# Autodesk Inventor assembly: Сборка
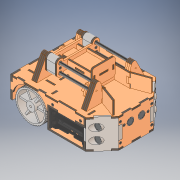
[picture p0: Inventor's stored thumbnail of the model, 180x180]
Saved by Autodesk Inventor 2019 (Build 230136000, 136)
## iProperties
Created: 2020-12-06
Part Number: Сборка
Material: Типовые
Document SubType Name: Assembly
Designer: Professional
Author: Professional
## Documents named in this file (51)
- C:\Users\Professional\Documents\DeliveryBot\3dModels\assembly.iam
- C:\Users\Professional\Documents\DeliveryBot\3dModels\Components\42BYGH47.ipt
- C:\Users\Professional\Documents\DeliveryBot\3dModels\LaserCutter\base.ipt
- C:\Users\Professional\Documents\DeliveryBot\3dModels\LaserCutter\top.ipt
- C:\Users\Professional\Documents\DeliveryBot\3dModels\LaserCutter\batTop.ipt
- C:\Users\Professional\Documents\DeliveryBot\3dModels\3DPrinter\Sensor_L.ipt
- C:\Users\Professional\Documents\DeliveryBot\3dModels\LaserCutter\batMain.ipt
- C:\Users\Professional\Documents\DeliveryBot\3dModels\LaserCutter\batBack.ipt
- C:\Users\Professional\Documents\DeliveryBot\3dModels\LaserCutter\batN.ipt
- C:\Users\Professional\Documents\DeliveryBot\3dModels\LaserCutter\spacer.ipt
- C:\Users\Professional\Documents\DeliveryBot\3dModels\LaserCutter\stepperMount.ipt
- C:\Users\Professional\Documents\DeliveryBot\3dModels\LaserCutter\stiffenerFront.ipt
- C:\Users\Professional\Documents\DeliveryBot\3dModels\LaserCutter\stiffenerBack.ipt
- C:\Users\Professional\Documents\DeliveryBot\3dModels\3DPrinter\sameSpacer.ipt
- C:\Users\Professional\Documents\DeliveryBot\3dModels\LaserCutter\back.ipt
- C:\Users\Professional\Documents\DeliveryBot\3dModels\3DPrinter\wheel_L.ipt
- C:\Users\Professional\Documents\DeliveryBot\3dModels\3DPrinter\wheel_R.ipt
- C:\Users\Professional\Documents\DeliveryBot\3dModels\LaserCutter\protector.ipt
- C:\Users\Professional\Documents\DeliveryBot\3dModels\components\HC-SR04.ipt
- C:\Users\Professional\Documents\DeliveryBot\3dModels\components\CNC shield.ipt
- C:\Users\Professional\Documents\DeliveryBot\3dModels\Components\2x18650 holder.ipt
- C:\Users\Professional\Documents\DeliveryBot\3dModels\components\smallWheel.ipt
- C:\Users\Professional\Documents\DeliveryBot\3dModels\3DPrinter\smallWheelStator.ipt
- C:\Users\Professional\Documents\DeliveryBot\3dModels\3DPrinter\CupHolder.ipt
- C:\Users\Professional\Documents\DeliveryBot\3dModels\Components\LineSensor.ipt
- C:\Users\Professional\Documents\DeliveryBot\3dModels\3DPrinter\StructureCenter.ipt
- C:\Users\Professional\Documents\DeliveryBot\3dModels\3DPrinter\CupHolderBack.ipt
- C:\Users\Professional\Documents\DeliveryBot\3dModels\3DPrinter\Sensor_R.ipt
- C:\Users\Professional\Documents\DeliveryBot\3dModels\LaserCutter\ElectronicPlate.ipt
- C:\Users\Professional\Documents\DeliveryBot\3dModels\Components\DC-DC sown.ipt
- C:\Users\Professional\Documents\DeliveryBot\3dModels\Fasteners\M3x16P.ipt
- C:\Users\Professional\Documents\DeliveryBot\3dModels\Fasteners\M3x10P.ipt
- C:\Users\Professional\Documents\DeliveryBot\3dModels\3DPrinter\FrontSensor.ipt
- C:\Users\Professional\Documents\DeliveryBot\3dModels\Components\ArduinoMega.ipt
- C:\Users\Professional\Documents\DeliveryBot\3dModels\LaserCutter\HolderDCDC.ipt
- C:\Users\Professional\Documents\DeliveryBot\3dModels\LaserCutter\stiffenerDCDC.ipt
- C:\Users\Professional\Documents\DeliveryBot\3dModels\Fasteners\M3_MF_6mm.ipt
- C:\Users\Professional\Documents\DeliveryBot\3dModels\LaserCutter\topCase.ipt
- C:\Users\Professional\Documents\DeliveryBot\3dModels\Components\SFC6.ipt
- C:\Users\Professional\Documents\DeliveryBot\3dModels\Components\LM6UU.ipt
- C:\Users\Professional\Documents\DeliveryBot\3dModels\LaserCutter\HolderSFC6.ipt
- C:\Users\Professional\Documents\DeliveryBot\3dModels\LaserCutter\StopperSFC6.ipt
- C:\Users\Professional\Documents\DeliveryBot\3dModels\LaserCutter\PistonPart1.ipt
- C:\Users\Professional\Documents\DeliveryBot\3dModels\LaserCutter\PistonPart2.ipt
- C:\Users\Professional\Documents\DeliveryBot\3dModels\LaserCutter\PistonPart3.ipt
- C:\Users\Professional\Documents\DeliveryBot\3dModels\LaserCutter\PistonPart4.ipt
- C:\Users\Professional\Documents\DeliveryBot\3dModels\LaserCutter\PistonPart5.ipt
- C:\Users\Professional\Documents\DeliveryBot\3dModels\3DPrinter\BearingIn.ipt
- C:\Users\Professional\Documents\DeliveryBot\3dModels\LaserCutter\Limiter1.ipt
- C:\Users\Professional\Documents\DeliveryBot\3dModels\LaserCutter\Limiter2.ipt
- C:\Users\Professional\Documents\DeliveryBot\3dModels\LaserCutter\Limiter3.ipt
## Components (164 placed, 50 different names)
1. 42BYGH47:1 — Угол:1, Жесткий:24, С поворотом:2
2. base:1 — Жесткий:1, Жесткий:4, Жесткий:6, Жесткий:8, Жесткий:9, Жесткий:10, Жесткий:11, Жесткий:12, Жесткий:18, Жесткий:19, Жесткий:22, Жесткий:23, Жесткий:37, Жесткий:38, Жесткий:45, Жесткий:46, С поворотом:4, С поворотом:5, С поворотом:31, С поворотом:32, С поворотом:33, С поворотом:34, С поворотом:65, С поворотом:74, С поворотом:75, С поворотом:76, С поворотом:77, С поворотом:90, С поворотом:91, С поворотом:92, С поворотом:93, С поворотом:94, С поворотом:95, С поворотом:96, С поворотом:97
3. top:1 — Жесткий:1, С поворотом:70, С поворотом:71, С поворотом:72, С поворотом:73, Жесткий:64, Жесткий:80, Жесткий:81, Жесткий:82
4. 42BYGH47:2 — Угол:1, Жесткий:25, С поворотом:1
5. batTop:1 — Жесткий:8, Жесткий:13, С поворотом:69
6. batTop:2 — Жесткий:4, Жесткий:15, Жесткий:51, С поворотом:10
7. Sensor_L:2 — Жесткий:6, Жесткий:33
8. batMain:1 — Жесткий:10, Жесткий:35
9. batMain:2 — Жесткий:9, Жесткий:53, Угол:4
10. batBack:1 — Жесткий:11, С поворотом:66
11. batBack:2 — Жесткий:12, С поворотом:9
12. batN:1 — Жесткий:13, Жесткий:16
13. batN:2 — Жесткий:15, Жесткий:28
14. spacer:1 — Жесткий:16, Жесткий:40, С поворотом:67, С поворотом:68
15. stepperMount:1 — Жесткий:19, Жесткий:24, С поворотом:27, С поворотом:28, С поворотом:29, С поворотом:30, С поворотом:78, С поворотом:79, С поворотом:80, С поворотом:81
16. stepperMount:2 — Жесткий:18, Жесткий:25, С поворотом:19, С поворотом:20, С поворотом:21, С поворотом:22, С поворотом:82, С поворотом:83, С поворотом:84, С поворотом:85
17. stiffenerFront:1 — Жесткий:22, Жесткий:47, Жесткий:48, С поворотом:15, С поворотом:16, С поворотом:17, С поворотом:18
18. stiffenerBack:1 — Жесткий:23, Жесткий:31, Жесткий:49, Жесткий:50, С поворотом:11, С поворотом:12, С поворотом:13, С поворотом:14
19. back:1 — Жесткий:29, Жесткий:30, Жесткий:39, С поворотом:23, С поворотом:24, С поворотом:25, С поворотом:26
20. wheel_L:2 — С поворотом:1
21. wheel_R:1 — С поворотом:2
22. spacer:2 — Жесткий:28, Жесткий:41, Жесткий:63, С поворотом:8
23. protector:1 — Жесткий:29
24. protector:2 — Жесткий:30
25. sameSpacer:1 — Жесткий:31, Жесткий:39
26. smallWheel:1 — С поворотом:3
27. smallWheelStator:1 — Жесткий:38, С поворотом:98
28. smallWheelStator:2 — Жесткий:37, С поворотом:3
29. CupHolder:1 — Жесткий:41
30. CupHolder:2 — Жесткий:40
31. StructureCenter:1 — Жесткий:48
32. StructureCenter:2 — Жесткий:47, Цилиндрический:1
33. CupHolderBack:1 — Жесткий:50
34. CupHolderBack:2 — Жесткий:49
35. Sensor_R:1 — Жесткий:51, Жесткий:52
36. FrontSensor:1 — Жесткий:64, Жесткий:65
37. topCase:1 — Жесткий:82, Жесткий:83, Жесткий:87, Жесткий:90, Жесткий:91, Угол:7, Угол:8, Жесткий:111, Жесткий:112, Жесткий:113, Жесткий:114, Жесткий:115
38. SFC6:1 — Жесткий:86, Цилиндрический:2
39. LM6UU:2 — Цилиндрический:2, Заподлицо:2
40. HolderSFC6:1 — Жесткий:83, Жесткий:84
41. HolderSFC6:2 — Жесткий:84, Жесткий:85, Жесткий:86, Жесткий:96
42. StopperSFC6:1 — Жесткий:85
43. StopperSFC6:3 — Жесткий:90, Жесткий:94
44. StopperSFC6:4 — Жесткий:87, Жесткий:88
45. HolderSFC6:3 — Жесткий:88, Жесткий:89
46. HolderSFC6:4 — Жесткий:89
47. StopperSFC6:5 — Жесткий:91, Жесткий:92
48. HolderSFC6:6 — Жесткий:92, Жесткий:93, Жесткий:97, Жесткий:98
49. HolderSFC6:7 — Жесткий:93
50. HolderSFC6:8 — Жесткий:95
51. HolderSFC6:9 — Жесткий:94, Жесткий:95
52. SFC6:4 — Жесткий:96
53. LM6UU:3 — Заподлицо:2, Заподлицо:3, Жесткий:99, Жесткий:105
54. SFC6:5 — Жесткий:98
55. LM6UU:4 — Заподлицо:1, Заподлицо:3, С поворотом:101
56. SFC6:6 — Жесткий:97
57. LM6UU:5 — Заподлицо:1
58. PistonPart1:1 — Жесткий:99, Угол:7, Жесткий:104, Жесткий:106, Жесткий:107, Жесткий:108
59. PistonPart2:1 — С поворотом:101, Угол:8, Жесткий:109, Жесткий:110
60. PistonPart3:1 — Жесткий:101, Жесткий:102, Жесткий:103, Жесткий:104
61. PistonPart4:1 — Жесткий:102
62. PistonPart4:2 — Жесткий:101
63. PistonPart5:1 — Жесткий:103
64. BearingIn:1 — Жесткий:106
65. BearingIn:2 — Жесткий:105
66. M3x10P:52 — Жесткий:107
67. M3x10P:53 — Жесткий:108
68. M3x10P:54 — Жесткий:109
69. M3x10P:55 — Жесткий:110
70. Limiter1:1 — Жесткий:111
71. Limiter1:2 — Жесткий:112
72. Limiter2:1 — Жесткий:113
73. Limiter3:1 — Жесткий:115
74. Limiter3:2 — Жесткий:114
75. M3x10P:42 — С поворотом:90
76. M3x10P:43 — С поворотом:92
77. M3x10P:44 — С поворотом:91
78. M3x10P:45 — С поворотом:93
79. M3x10P:46 — С поворотом:97
80. M3x10P:47 — С поворотом:94
81. M3x10P:48 — С поворотом:96
82. M3x10P:49 — С поворотом:95
83. M3x16P:16 — С поворотом:98
84. M3x10P:50 — Жесткий:80
85. M3x10P:51 — Жесткий:81
86. M3x16P:2 — С поворотом:8
87. M3x16P:3 — С поворотом:9
88. M3x16P:5 — С поворотом:10
89. M3x16P:6 — С поворотом:14
90. M3x16P:7 — С поворотом:13
91. M3x16P:8 — С поворотом:12
92. M3x16P:11 — С поворотом:11
93. M3x10P:2 — С поворотом:16
94. M3x10P:3 — С поворотом:17
95. M3x10P:4 — С поворотом:15
96. M3x10P:5 — С поворотом:21
97. M3x10P:6 — С поворотом:29
98. M3x10P:7 — С поворотом:23
99. M3x10P:8 — С поворотом:22
100. M3x10P:9 — С поворотом:27
101. M3x10P:10 — С поворотом:28
102. M3x10P:11 — С поворотом:19
103. M3x10P:12 — С поворотом:30
104. M3x10P:13 — С поворотом:31
105. M3x10P:14 — С поворотом:20
106. M3x10P:15 — С поворотом:26
107. M3x10P:16 — С поворотом:24
108. M3x10P:17 — С поворотом:25
109. M3x10P:18 — С поворотом:32
110. M3x10P:19 — С поворотом:34
111. M3x10P:20 — С поворотом:33
112. M3x10P:21 — С поворотом:65
113. M3x16P:12 — С поворотом:68
114. M3x16P:13 — С поворотом:67
115. M3x16P:14 — С поворотом:69
116. M3x16P:15 — С поворотом:66
117. M3x10P:22 — С поворотом:73
118. M3x10P:23 — С поворотом:72
119. M3x10P:24 — С поворотом:71
120. M3x10P:25 — С поворотом:70
121. M3x10P:26 — С поворотом:74
122. M3x10P:27 — С поворотом:75
123. M3x10P:28 — С поворотом:76
124. M3x10P:29 — С поворотом:77
125. M3x10P:30 — С поворотом:81
126. M3x10P:31 — С поворотом:80
127. M3x10P:32 — С поворотом:79
128. M3x10P:33 — С поворотом:78
129. M3x10P:34 — С поворотом:82
130. M3x10P:35 — С поворотом:83
131. M3x10P:36 — С поворотом:84
132. M3x10P:37 — С поворотом:85
133. M3x10P:1 — С поворотом:18
134. M3x16P:1 — Жесткий:63
135. HolderDCDC:1 — Жесткий:66, Жесткий:67, Жесткий:68, Жесткий:69, Жесткий:70, Жесткий:71, Жесткий:72
136. stiffenerDCDC:1 — Жесткий:67
137. stiffenerDCDC:2 — Жесткий:68
138. DC-DC sown:1 — Жесткий:73
139. ArduinoMega:1 — С поворотом:99, Угол:5, С поворотом:100, Угол:6
140. CNC shield:1 — С поворотом:100, Угол:6
141. ElectronicPlate:1 — Цилиндрический:1, С поворотом:86, С поворотом:87, С поворотом:88, С поворотом:89, Жесткий:66, Угол:4, Жесткий:74, Жесткий:75, Жесткий:76, Жесткий:77, Жесткий:78, Жесткий:79, Угол:5
142. M3x10P:38 — С поворотом:87
143. M3x10P:39 — С поворотом:89
144. M3x10P:40 — С поворотом:88
145. M3x10P:41 — С поворотом:86
146. M3_MF_6mm:1 — Жесткий:69, Жесткий:73
147. M3_MF_6mm:2 — Жесткий:70
148. M3_MF_6mm:3 — Жесткий:72
149. M3_MF_6mm:4 — Жесткий:71
150. M3_MF_6mm:5 — Жесткий:76
151. M3_MF_6mm:6 — Жесткий:75
152. M3_MF_6mm:7 — Жесткий:77
153. M3_MF_6mm:8 — Жесткий:78
154. M3_MF_6mm:9 — Жесткий:74, С поворотом:99
155. M3_MF_6mm:10 — Жесткий:79
156. 2x18650 holder:2 — Жесткий:53
157. HC-SR04:2 — Жесткий:52
158. HC-SR04:1 — Жесткий:33
159. 2x18650 holder:1 — Жесткий:35
160. LineSensor:4 — С поворотом:4
161. LineSensor:3 — С поворотом:5
162. LineSensor:2 — Жесткий:45
163. LineSensor:1 — Жесткий:46
164. HC-SR04:3 — Жесткий:65
## Relationships (172: WeldJoint 89, RevoluteJoint 69, Angle 6, CylindricalJoint 5, Flush 3)
- Жесткий:1 [WeldJoint]: base:1 ↔ top:1
- Угол:1 [Angle] (180 deg): 42BYGH47:1 ↔ 42BYGH47:2
- Жесткий:4 [WeldJoint]: base:1 ↔ batTop:2
- Жесткий:6 [WeldJoint]: base:1 ↔ Sensor_L:2
- Жесткий:8 [WeldJoint]: base:1 ↔ batTop:1
- Жесткий:9 [WeldJoint]: base:1 ↔ batMain:2
- Жесткий:10 [WeldJoint]: base:1 ↔ batMain:1
- Жесткий:11 [WeldJoint]: base:1 ↔ batBack:1
- Жесткий:12 [WeldJoint]: base:1 ↔ batBack:2
- Жесткий:13 [WeldJoint]: batTop:1 ↔ batN:1
- Жесткий:15 [WeldJoint]: batTop:2 ↔ batN:2
- Жесткий:16 [WeldJoint]: batN:1 ↔ spacer:1
- Жесткий:18 [WeldJoint]: base:1 ↔ stepperMount:2
- Жесткий:19 [WeldJoint]: base:1 ↔ stepperMount:1
- Жесткий:22 [WeldJoint]: base:1 ↔ stiffenerFront:1
- Жесткий:23 [WeldJoint]: base:1 ↔ stiffenerBack:1
- Жесткий:24 [WeldJoint]: 42BYGH47:1 ↔ stepperMount:1
- Жесткий:25 [WeldJoint]: 42BYGH47:2 ↔ stepperMount:2
- С поворотом:1 [RevoluteJoint] (-19 mm): 42BYGH47:2 ↔ wheel_L:2
- С поворотом:2 [RevoluteJoint] (-19 mm): 42BYGH47:1 ↔ wheel_R:1
- Жесткий:28 [WeldJoint]: batN:2 ↔ spacer:2
- Жесткий:29 [WeldJoint]: back:1 ↔ protector:1
- Жесткий:30 [WeldJoint]: back:1 ↔ protector:2
- Жесткий:31 [WeldJoint]: stiffenerBack:1 ↔ sameSpacer:1
- Жесткий:33 [WeldJoint]: Sensor_L:2 ↔ HC-SR04:1
- Жесткий:35 [WeldJoint]: batMain:1 ↔ 2x18650 holder:1
- Жесткий:37 [WeldJoint]: base:1 ↔ smallWheelStator:2
- Жесткий:38 [WeldJoint]: base:1 ↔ smallWheelStator:1
- С поворотом:3 [RevoluteJoint]: smallWheel:1 ↔ smallWheelStator:2
- Жесткий:39 [WeldJoint]: back:1 ↔ sameSpacer:1
- Жесткий:40 [WeldJoint]: spacer:1 ↔ CupHolder:2
- Жесткий:41 [WeldJoint]: spacer:2 ↔ CupHolder:1
- Жесткий:45 [WeldJoint]: base:1 ↔ LineSensor:2
- Жесткий:46 [WeldJoint]: base:1 ↔ LineSensor:1
- С поворотом:4 [RevoluteJoint]: base:1 ↔ LineSensor:4
- С поворотом:5 [RevoluteJoint]: base:1 ↔ LineSensor:3
- Жесткий:47 [WeldJoint]: stiffenerFront:1 ↔ StructureCenter:2
- Жесткий:48 [WeldJoint]: stiffenerFront:1 ↔ StructureCenter:1
- Жесткий:49 [WeldJoint]: stiffenerBack:1 ↔ CupHolderBack:2
- Жесткий:50 [WeldJoint]: stiffenerBack:1 ↔ CupHolderBack:1
- Жесткий:51 [WeldJoint]: batTop:2 ↔ Sensor_R:1
- Жесткий:52 [WeldJoint]: Sensor_R:1 ↔ HC-SR04:2
- Жесткий:53 [WeldJoint]: batMain:2 ↔ 2x18650 holder:2
- Цилиндрический:1 [CylindricalJoint]: StructureCenter:2 ↔ ElectronicPlate:1
- Жесткий:63 [WeldJoint]: spacer:2 ↔ M3x16P:1
- С поворотом:8 [RevoluteJoint]: spacer:2 ↔ M3x16P:2
- С поворотом:9 [RevoluteJoint]: batBack:2 ↔ M3x16P:3
- С поворотом:10 [RevoluteJoint]: batTop:2 ↔ M3x16P:5
- С поворотом:11 [RevoluteJoint]: stiffenerBack:1 ↔ M3x16P:11
- С поворотом:12 [RevoluteJoint]: stiffenerBack:1 ↔ M3x16P:8
- С поворотом:13 [RevoluteJoint]: stiffenerBack:1 ↔ M3x16P:7
- С поворотом:14 [RevoluteJoint]: stiffenerBack:1 ↔ M3x16P:6
- С поворотом:15 [RevoluteJoint]: stiffenerFront:1 ↔ M3x10P:4
- С поворотом:16 [RevoluteJoint]: stiffenerFront:1 ↔ M3x10P:2
- С поворотом:17 [RevoluteJoint]: stiffenerFront:1 ↔ M3x10P:3
- С поворотом:18 [RevoluteJoint]: stiffenerFront:1 ↔ M3x10P:1
- С поворотом:19 [RevoluteJoint]: stepperMount:2 ↔ M3x10P:11
- С поворотом:20 [RevoluteJoint]: stepperMount:2 ↔ M3x10P:14
- С поворотом:21 [RevoluteJoint]: stepperMount:2 ↔ M3x10P:5
- С поворотом:22 [RevoluteJoint]: stepperMount:2 ↔ M3x10P:8
- С поворотом:23 [RevoluteJoint]: back:1 ↔ M3x10P:7
- С поворотом:24 [RevoluteJoint]: back:1 ↔ M3x10P:16
- С поворотом:25 [RevoluteJoint]: back:1 ↔ M3x10P:17
- С поворотом:26 [RevoluteJoint]: back:1 ↔ M3x10P:15
- С поворотом:27 [RevoluteJoint]: stepperMount:1 ↔ M3x10P:9
- С поворотом:28 [RevoluteJoint]: stepperMount:1 ↔ M3x10P:10
- С поворотом:29 [RevoluteJoint]: stepperMount:1 ↔ M3x10P:6
- С поворотом:30 [RevoluteJoint]: stepperMount:1 ↔ M3x10P:12
- С поворотом:31 [RevoluteJoint]: base:1 ↔ M3x10P:13
- С поворотом:32 [RevoluteJoint]: base:1 ↔ M3x10P:18
- С поворотом:33 [RevoluteJoint]: base:1 ↔ M3x10P:20
- С поворотом:34 [RevoluteJoint]: base:1 ↔ M3x10P:19
- С поворотом:65 [RevoluteJoint]: base:1 ↔ M3x10P:21
- С поворотом:66 [RevoluteJoint]: batBack:1 ↔ M3x16P:15
- С поворотом:67 [RevoluteJoint]: spacer:1 ↔ M3x16P:13
- С поворотом:68 [RevoluteJoint]: spacer:1 ↔ M3x16P:12
- С поворотом:69 [RevoluteJoint]: batTop:1 ↔ M3x16P:14
- С поворотом:70 [RevoluteJoint]: top:1 ↔ M3x10P:25
- С поворотом:71 [RevoluteJoint]: top:1 ↔ M3x10P:24
- С поворотом:72 [RevoluteJoint]: top:1 ↔ M3x10P:23
- С поворотом:73 [RevoluteJoint]: top:1 ↔ M3x10P:22
- С поворотом:74 [RevoluteJoint]: base:1 ↔ M3x10P:26
- С поворотом:75 [RevoluteJoint]: base:1 ↔ M3x10P:27
- С поворотом:76 [RevoluteJoint]: base:1 ↔ M3x10P:28
- С поворотом:77 [RevoluteJoint]: base:1 ↔ M3x10P:29
- С поворотом:78 [RevoluteJoint]: stepperMount:1 ↔ M3x10P:33
- С поворотом:79 [RevoluteJoint]: stepperMount:1 ↔ M3x10P:32
- С поворотом:80 [RevoluteJoint]: stepperMount:1 ↔ M3x10P:31
- С поворотом:81 [RevoluteJoint]: stepperMount:1 ↔ M3x10P:30
- С поворотом:82 [RevoluteJoint]: stepperMount:2 ↔ M3x10P:34
- С поворотом:83 [RevoluteJoint]: stepperMount:2 ↔ M3x10P:35
- С поворотом:84 [RevoluteJoint]: stepperMount:2 ↔ M3x10P:36
- С поворотом:85 [RevoluteJoint]: stepperMount:2 ↔ M3x10P:37
- С поворотом:86 [RevoluteJoint]: ElectronicPlate:1 ↔ M3x10P:41
- С поворотом:87 [RevoluteJoint]: ElectronicPlate:1 ↔ M3x10P:38
- С поворотом:88 [RevoluteJoint]: ElectronicPlate:1 ↔ M3x10P:40
- С поворотом:89 [RevoluteJoint]: ElectronicPlate:1 ↔ M3x10P:39
- С поворотом:90 [RevoluteJoint]: base:1 ↔ M3x10P:42
- С поворотом:91 [RevoluteJoint]: base:1 ↔ M3x10P:44
- С поворотом:92 [RevoluteJoint]: base:1 ↔ M3x10P:43
- С поворотом:93 [RevoluteJoint]: base:1 ↔ M3x10P:45
- С поворотом:94 [RevoluteJoint]: base:1 ↔ M3x10P:47
- С поворотом:95 [RevoluteJoint]: base:1 ↔ M3x10P:49
- С поворотом:96 [RevoluteJoint]: base:1 ↔ M3x10P:48
- С поворотом:97 [RevoluteJoint]: base:1 ↔ M3x10P:46
- С поворотом:98 [RevoluteJoint]: smallWheelStator:1 ↔ M3x16P:16
- Жесткий:64 [WeldJoint]: top:1 ↔ FrontSensor:1
- Жесткий:65 [WeldJoint]: FrontSensor:1 ↔ HC-SR04:3
- Жесткий:66 [WeldJoint]: HolderDCDC:1 ↔ ElectronicPlate:1
- Жесткий:67 [WeldJoint]: HolderDCDC:1 ↔ stiffenerDCDC:1
- Жесткий:68 [WeldJoint]: HolderDCDC:1 ↔ stiffenerDCDC:2
- Угол:4 [Angle] (180 deg): batMain:2 ↔ ElectronicPlate:1
- Жесткий:69 [WeldJoint]: HolderDCDC:1 ↔ M3_MF_6mm:1
- Жесткий:70 [WeldJoint]: HolderDCDC:1 ↔ M3_MF_6mm:2
- Жесткий:71 [WeldJoint]: HolderDCDC:1 ↔ M3_MF_6mm:4
- Жесткий:72 [WeldJoint]: HolderDCDC:1 ↔ M3_MF_6mm:3
- Жесткий:73 [WeldJoint]: DC-DC sown:1 ↔ M3_MF_6mm:1
- Жесткий:74 [WeldJoint]: ElectronicPlate:1 ↔ M3_MF_6mm:9
- Жесткий:75 [WeldJoint]: ElectronicPlate:1 ↔ M3_MF_6mm:6
- Жесткий:76 [WeldJoint]: ElectronicPlate:1 ↔ M3_MF_6mm:5
- Жесткий:77 [WeldJoint]: ElectronicPlate:1 ↔ M3_MF_6mm:7
- Жесткий:78 [WeldJoint]: ElectronicPlate:1 ↔ M3_MF_6mm:8
- Жесткий:79 [WeldJoint]: ElectronicPlate:1 ↔ M3_MF_6mm:10
- С поворотом:99 [RevoluteJoint]: ArduinoMega:1 ↔ M3_MF_6mm:9
- Угол:5 [Angle] (0 deg): ArduinoMega:1 ↔ ElectronicPlate:1
- С поворотом:100 [RevoluteJoint]: ArduinoMega:1 ↔ CNC shield:1
- Угол:6 [Angle] (0 deg): ArduinoMega:1 ↔ CNC shield:1
- Жесткий:80 [WeldJoint]: top:1 ↔ M3x10P:50
- Жесткий:81 [WeldJoint]: top:1 ↔ M3x10P:51
- Жесткий:82 [WeldJoint]: top:1 ↔ topCase:1
- Жесткий:83 [WeldJoint]: topCase:1 ↔ HolderSFC6:1
- Жесткий:84 [WeldJoint]: HolderSFC6:1 ↔ HolderSFC6:2
- Жесткий:85 [WeldJoint]: HolderSFC6:2 ↔ StopperSFC6:1
- Жесткий:86 [WeldJoint]: SFC6:1 ↔ HolderSFC6:2
- Жесткий:87 [WeldJoint]: topCase:1 ↔ StopperSFC6:4
- Жесткий:88 [WeldJoint]: StopperSFC6:4 ↔ HolderSFC6:3
- Жесткий:89 [WeldJoint]: HolderSFC6:3 ↔ HolderSFC6:4
- Жесткий:90 [WeldJoint]: topCase:1 ↔ StopperSFC6:3
- Жесткий:91 [WeldJoint]: topCase:1 ↔ StopperSFC6:5
- Жесткий:92 [WeldJoint]: StopperSFC6:5 ↔ HolderSFC6:6
- Жесткий:93 [WeldJoint]: HolderSFC6:6 ↔ HolderSFC6:7
- Жесткий:94 [WeldJoint]: StopperSFC6:3 ↔ HolderSFC6:9
- Жесткий:95 [WeldJoint]: HolderSFC6:8 ↔ HolderSFC6:9
- Цилиндрический:2 [CylindricalJoint]: SFC6:1 ↔ LM6UU:2
- [CylindricalJoint]: SFC6:4 ↔ LM6UU:3
- [CylindricalJoint]: SFC6:5 ↔ LM6UU:4
- [CylindricalJoint]: SFC6:6 ↔ LM6UU:5
- Жесткий:96 [WeldJoint]: HolderSFC6:2 ↔ SFC6:4
- Жесткий:97 [WeldJoint]: HolderSFC6:6 ↔ SFC6:6
- Жесткий:98 [WeldJoint]: HolderSFC6:6 ↔ SFC6:5
- Заподлицо:1 [Flush]: LM6UU:4 ↔ LM6UU:5
- Заподлицо:2 [Flush]: LM6UU:2 ↔ LM6UU:3
- Заподлицо:3 [Flush]: LM6UU:3 ↔ LM6UU:4
- Жесткий:99 [WeldJoint]: LM6UU:3 ↔ PistonPart1:1
- Угол:7 [Angle] (0 deg): topCase:1 ↔ PistonPart1:1
- С поворотом:101 [RevoluteJoint]: LM6UU:4 ↔ PistonPart2:1
- Угол:8 [Angle] (0 deg): topCase:1 ↔ PistonPart2:1
- Жесткий:101 [WeldJoint]: PistonPart3:1 ↔ PistonPart4:2
- Жесткий:102 [WeldJoint]: PistonPart3:1 ↔ PistonPart4:1
- Жесткий:103 [WeldJoint]: PistonPart3:1 ↔ PistonPart5:1
- Жесткий:104 [WeldJoint]: PistonPart1:1 ↔ PistonPart3:1
- Жесткий:105 [WeldJoint]: LM6UU:3 ↔ BearingIn:2
- Жесткий:106 [WeldJoint]: PistonPart1:1 ↔ BearingIn:1
- Жесткий:107 [WeldJoint]: PistonPart1:1 ↔ M3x10P:52
- Жесткий:108 [WeldJoint]: PistonPart1:1 ↔ M3x10P:53
- Жесткий:109 [WeldJoint]: PistonPart2:1 ↔ M3x10P:54
- Жесткий:110 [WeldJoint]: PistonPart2:1 ↔ M3x10P:55
- Жесткий:111 [WeldJoint]: topCase:1 ↔ Limiter1:1
- Жесткий:112 [WeldJoint]: topCase:1 ↔ Limiter1:2
- Жесткий:113 [WeldJoint]: topCase:1 ↔ Limiter2:1
- Жесткий:114 [WeldJoint]: topCase:1 ↔ Limiter3:2
- Жесткий:115 [WeldJoint]: topCase:1 ↔ Limiter3:1
## Named parameters: d275_d271 = 26.87744 deg, d276_d272 = -91 mm, d277_d273 = -12.00003 mm, d278_d274 = -8 mm, d279_d275_d271 = -21.136236 deg, d280_d276_d272 = -91 mm, d281_d277_d273 = -12.00003 mm, d282_d278_d274 = -8 mm, d283_d275_d271 = -80.895457 deg, d284_d276_d272 = -91 mm, d285_d277_d273 = -12.00003 mm, d286_d278_d274 = -8 mm
